# Autodesk Inventor assembly: Assembly6
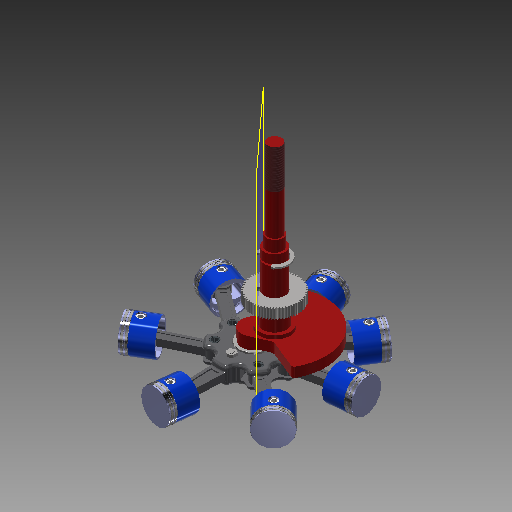
[picture p0: Inventor's stored thumbnail of the model, 512x512]
Saved by Autodesk Inventor 2018 (Build 220112000, 112)
## iProperties
Created: 2023-04-24
Part Number: Assembly6
Document SubType Name: Assembly
Designer: Habib Mohamed
Author: Habib Mohamed
## Documents named in this file (15)
- D:\Inventor\My projects\Rotary Engine\Assembly\Assembly6(Piston Sub Assembly Major).iam
- D:\Inventor\My projects\Rotary Engine\Component 2 (Connecting Rod Hub).ipt
- D:\Inventor\My projects\Rotary Engine\Component 31(Rod Axle).ipt
- D:\Inventor\My projects\Rotary Engine\Assembly\Assembly4 (Piston Sub Assembly Shrunk).iam
- D:\Inventor\My projects\Rotary Engine\Shaft.ipt
- D:\Inventor\My projects\Rotary Engine\Component 16 (Sun Wheel).ipt
- D:\Inventor\My projects\Rotary Engine\Component 17 (Feather Key).ipt
- D:\Inventor\My projects\Rotary Engine\Component 7 (Cover Plate).ipt
- C:\Users\Habib Mohamed\Documents\Inventor\Content Center Files\R2018\en-US\DIN 617 SKF(2)\DIN 617 SKF - SKF NA 4900 RS.ipt
- C:\Users\Habib Mohamed\Documents\Inventor\Content Center Files\R2018\en-US\DIN 6799\DIN 6799 - 9 10.ipt
- C:\Users\Habib Mohamed\Documents\Inventor\Content Center Files\R2018\en-US\DIN 6799\DIN 6799 - 10 11.ipt
- D:\Inventor\My projects\Rotary Engine\Assembly\Assembly6\Design Accelerator\Bolted Connection1.iam
- D:\Inventor\My projects\Rotary Engine\Assembly\Assembly6\Design Accelerator\Bolted Connection2.iam
- C:\Users\Habib Mohamed\Documents\Inventor\Content Center Files\R2018\en-US\DIN EN 24 036(2)\DIN EN 24 036 - M3.ipt
- D:\Inventor\My projects\Rotary Engine\Component 6 (Connecting Rod).ipt
## Components (31 placed, 13 different names)
1. Component 2 (Connecting Rod Hub):1 — Mate:1, Mate:2, Mate:15, Mate:16, Mate:17, Mate:18, Mate:19, Mate:20, Flush:1, Flush:2, Flush:3, Flush:4, Flush:5, Mate:21, Mate:22, Mate:29, Mate:30, Flush:6, Mate:33, Mate:34, Mate:40, Mate:42, Mate:44, Mate:46, Mate:61, Mate:62, Mate:63, Mate:64, Mate:65, Mate:66
2. Component 31(Rod Axle):1 — Mate:18, Flush:1, Mate:56
3. Assembly4 (Piston Sub Assembly Shrunk):1 [sub-assembly] — Mate:21, Mate:22
4. Component 31(Rod Axle):2 — Mate:16, Flush:3, Mate:58
5. Component 31(Rod Axle):3 — Mate:15, Flush:2, Mate:57
6. Component 31(Rod Axle):4 — Mate:20, Flush:5, Mate:60
7. Component 31(Rod Axle):5 — Mate:19, Flush:4, Mate:59
8. Component 31(Rod Axle):6 — Mate:17, Mate:55
9. Shaft:1 — Mate:23, Mate:24, Mate:25, Mate:26, Mate:27, Mate:28, Mate:29, Mate:31, Mate:32, Mate:35, Mate:37, Mate:38
10. Component 16 (Sun Wheel):1 — Mate:26, Mate:27, Mate:28
11. Component 17 (Feather Key):1 — Mate:23, Mate:24, Mate:25
12. Component 7 (Cover Plate):1 — Mate:32, Mate:33, Mate:34, Mate:36, Mate:39, Mate:41
13. DIN 617 SKF- with Inner Ring - NA 49...RS SKF NA 4900 RS:1 — Mate:30, Mate:31, Flush:6
14. DIN 6799 9:1 — Mate:35, Mate:36
15. DIN 6799 10:1 — Mate:37, Mate:38
16. Bolted Connection:1 [sub-assembly] — Mate:39, Mate:40, Mate:45
17. Bolted Connection:2 [sub-assembly] — Mate:41, Mate:42, Mate:43
18. DIN EN 24036 M3:1 — Mate:43, Mate:44
19. DIN EN 24036 M3:2 — Mate:45, Mate:46
20. Assembly4 (Piston Sub Assembly Shrunk):2 [sub-assembly] — Mate:47, Flush:10
21. Assembly4 (Piston Sub Assembly Shrunk):3 [sub-assembly] — Mate:48, Flush:9
22. Assembly4 (Piston Sub Assembly Shrunk):4 [sub-assembly] — Mate:49, Flush:8
23. Assembly4 (Piston Sub Assembly Shrunk):5 [sub-assembly] — Mate:50, Flush:7
24. Assembly4 (Piston Sub Assembly Shrunk):6 [sub-assembly] — Mate:51, Mate:54
25. Assembly4 (Piston Sub Assembly Shrunk):7 [sub-assembly] — Mate:52, Mate:53
26. Component 6 (Connecting Rod):1 — Mate:47, Flush:10, Mate:58, Mate:63
27. Component 6 (Connecting Rod):2 — Mate:48, Flush:9, Mate:59, Mate:62
28. Component 6 (Connecting Rod):3 — Mate:49, Flush:8, Mate:60, Mate:61
29. Component 6 (Connecting Rod):4 — Mate:50, Flush:7, Mate:57, Mate:64
30. Component 6 (Connecting Rod):5 — Mate:51, Mate:54, Mate:56, Mate:65
31. Component 6 (Connecting Rod):6 — Mate:52, Mate:53, Mate:55, Mate:66
## Relationships (64: Mate 54, Flush 10)
- Mate:1: Component 2 (Connecting Rod Hub):1
- Mate:2: Component 2 (Connecting Rod Hub):1
- Mate:15: Component 2 (Connecting Rod Hub):1 ↔ Component 31(Rod Axle):3
- Mate:16: Component 2 (Connecting Rod Hub):1 ↔ Component 31(Rod Axle):2
- Mate:17: Component 2 (Connecting Rod Hub):1 ↔ Component 31(Rod Axle):6
- Mate:18: Component 2 (Connecting Rod Hub):1 ↔ Component 31(Rod Axle):1
- Mate:19: Component 2 (Connecting Rod Hub):1 ↔ Component 31(Rod Axle):5
- Mate:20: Component 2 (Connecting Rod Hub):1 ↔ Component 31(Rod Axle):4
- Flush:1: Component 2 (Connecting Rod Hub):1 ↔ Component 31(Rod Axle):1
- Flush:2: Component 2 (Connecting Rod Hub):1 ↔ Component 31(Rod Axle):3
- Flush:3: Component 2 (Connecting Rod Hub):1 ↔ Component 31(Rod Axle):2
- Flush:4: Component 2 (Connecting Rod Hub):1 ↔ Component 31(Rod Axle):5
- Flush:5: Component 2 (Connecting Rod Hub):1 ↔ Component 31(Rod Axle):4
- Mate:21: Component 2 (Connecting Rod Hub):1 ↔ Assembly4 (Piston Sub Assembly Shrunk):1
- Mate:22: Component 2 (Connecting Rod Hub):1 ↔ Assembly4 (Piston Sub Assembly Shrunk):1
- Mate:23: Shaft:1 ↔ Component 17 (Feather Key):1
- Mate:24: Shaft:1 ↔ Component 17 (Feather Key):1
- Mate:25: Shaft:1 ↔ Component 17 (Feather Key):1
- Mate:26: Shaft:1 ↔ Component 16 (Sun Wheel):1
- Mate:27: Shaft:1 ↔ Component 16 (Sun Wheel):1
- Mate:28: Shaft:1 ↔ Component 16 (Sun Wheel):1
- Mate:29: Component 2 (Connecting Rod Hub):1 ↔ Shaft:1
- Mate:30: Component 2 (Connecting Rod Hub):1 ↔ DIN 617 SKF- with Inner Ring - NA 49...RS SKF NA 4900 RS:1
- Mate:31: Shaft:1 ↔ DIN 617 SKF- with Inner Ring - NA 49...RS SKF NA 4900 RS:1
- Flush:6: Component 2 (Connecting Rod Hub):1 ↔ DIN 617 SKF- with Inner Ring - NA 49...RS SKF NA 4900 RS:1
- Mate:32: Shaft:1 ↔ Component 7 (Cover Plate):1
- Mate:33: Component 2 (Connecting Rod Hub):1 ↔ Component 7 (Cover Plate):1
- Mate:34: Component 2 (Connecting Rod Hub):1 ↔ Component 7 (Cover Plate):1
- Mate:35: Shaft:1 ↔ DIN 6799 9:1
- Mate:36: Component 7 (Cover Plate):1 ↔ DIN 6799 9:1
- Mate:37: Shaft:1 ↔ DIN 6799 10:1
- Mate:38: Shaft:1 ↔ DIN 6799 10:1
- Mate:39: Component 7 (Cover Plate):1 ↔ Bolted Connection:1
- Mate:40: Component 2 (Connecting Rod Hub):1 ↔ Bolted Connection:1
- Mate:41: Component 7 (Cover Plate):1 ↔ Bolted Connection:2
- Mate:42: Component 2 (Connecting Rod Hub):1 ↔ Bolted Connection:2
- Mate:43: Bolted Connection:2 ↔ DIN EN 24036 M3:1
- Mate:44: Component 2 (Connecting Rod Hub):1 ↔ DIN EN 24036 M3:1
- Mate:45: Bolted Connection:1 ↔ DIN EN 24036 M3:2
- Mate:46: Component 2 (Connecting Rod Hub):1 ↔ DIN EN 24036 M3:2
- Mate:47: Assembly4 (Piston Sub Assembly Shrunk):2 ↔ Component 6 (Connecting Rod):1
- Mate:48: Assembly4 (Piston Sub Assembly Shrunk):3 ↔ Component 6 (Connecting Rod):2
- Mate:49: Assembly4 (Piston Sub Assembly Shrunk):4 ↔ Component 6 (Connecting Rod):3
- Mate:50: Assembly4 (Piston Sub Assembly Shrunk):5 ↔ Component 6 (Connecting Rod):4
- Mate:51: Assembly4 (Piston Sub Assembly Shrunk):6 ↔ Component 6 (Connecting Rod):5
- Mate:52: Assembly4 (Piston Sub Assembly Shrunk):7 ↔ Component 6 (Connecting Rod):6
- Mate:53: Assembly4 (Piston Sub Assembly Shrunk):7 ↔ Component 6 (Connecting Rod):6
- Mate:54: Assembly4 (Piston Sub Assembly Shrunk):6 ↔ Component 6 (Connecting Rod):5
- Flush:7: Assembly4 (Piston Sub Assembly Shrunk):5 ↔ Component 6 (Connecting Rod):4
- Flush:8: Assembly4 (Piston Sub Assembly Shrunk):4 ↔ Component 6 (Connecting Rod):3
- Flush:9: Assembly4 (Piston Sub Assembly Shrunk):3 ↔ Component 6 (Connecting Rod):2
- Flush:10: Assembly4 (Piston Sub Assembly Shrunk):2 ↔ Component 6 (Connecting Rod):1
- Mate:55: Component 31(Rod Axle):6 ↔ Component 6 (Connecting Rod):6
- Mate:56: Component 31(Rod Axle):1 ↔ Component 6 (Connecting Rod):5
- Mate:57: Component 31(Rod Axle):3 ↔ Component 6 (Connecting Rod):4
- Mate:58: Component 31(Rod Axle):2 ↔ Component 6 (Connecting Rod):1
- Mate:59: Component 31(Rod Axle):5 ↔ Component 6 (Connecting Rod):2
- Mate:60: Component 31(Rod Axle):4 ↔ Component 6 (Connecting Rod):3
- Mate:61: Component 2 (Connecting Rod Hub):1 ↔ Component 6 (Connecting Rod):3
- Mate:62: Component 2 (Connecting Rod Hub):1 ↔ Component 6 (Connecting Rod):2
- Mate:63: Component 2 (Connecting Rod Hub):1 ↔ Component 6 (Connecting Rod):1
- Mate:64: Component 2 (Connecting Rod Hub):1 ↔ Component 6 (Connecting Rod):4
- Mate:65: Component 2 (Connecting Rod Hub):1 ↔ Component 6 (Connecting Rod):5
- Mate:66: Component 2 (Connecting Rod Hub):1 ↔ Component 6 (Connecting Rod):6
